# Autodesk Inventor assembly: Assembly2
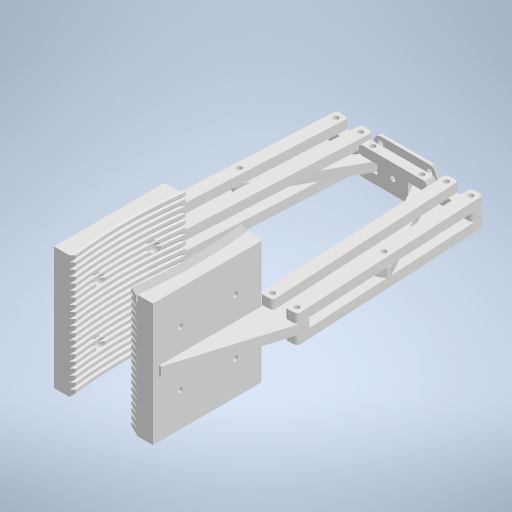
[picture p0: Inventor's stored thumbnail of the model, 512x512]
Saved by Autodesk Inventor 2023 (Build 270158000, 158)
## iProperties
Created: 2023-02-27
Part Number: Assembly2
Document SubType Name: Assembly
Designer: Gabriel - T3 CAD
Author: Gabriel - T3 CAD
## Documents named in this file (14)
- C:\Users\Gabriel - T3 CAD\Downloads\New folder\Assembly2.iam
- C:\Users\Gabriel - T3 CAD\Downloads\New folder\Outer swing.ipt
- C:\Users\Gabriel - T3 CAD\Downloads\New folder\Inner swing.ipt
- C:\Users\Gabriel - T3 CAD\Downloads\New folder\Pusher.ipt
- C:\Users\Gabriel - T3 CAD\Downloads\New folder\Connector.ipt
- C:\Users\Gabriel - T3 CAD\Downloads\New folder\Gripper triangle.ipt
- C:\Users\Gabriel - T3 CAD\Downloads\New folder\Gripper plate.ipt
- C:\Users\Gabriel - T3 CAD\Downloads\New folder\Outer swing_MIR.ipt
- C:\Users\Gabriel - T3 CAD\Downloads\New folder\Inner swing_MIR.ipt
- C:\Users\Gabriel - T3 CAD\Downloads\New folder\Pusher_MIR.ipt
- C:\Users\Gabriel - T3 CAD\Downloads\New folder\Gripper triangle_MIR.ipt
- C:\Users\Gabriel - T3 CAD\Downloads\New folder\Gripper plate_MIR.ipt
- C:\Users\Gabriel - T3 CAD\Downloads\New folder\Face Plate.ipt
- C:\Users\Gabriel - T3 CAD\Documents\GitHub\T3-CAD\Current Season CAD\Swerve-DriveTrain-V2.1 (LongBot)\Potential new gripper\Gripper plate v2.ipt
## Components (18 placed, 13 different names)
1. Outer swing:1 — Insert:1, Insert:7
2. Inner swing:1 — Insert:9, Insert:19
3. Pusher:1 — Insert:1, Insert:2, Insert:3
4. Outer swing:2 — Insert:2, Insert:8, Insert:23
5. Connector:1 — Insert:3, Insert:18, Insert:29
6. Inner swing:2 — Insert:10, Insert:20
7. Gripper triangle:1 — Rigid:1, Insert:7, Insert:8, Insert:9, Insert:10
8. Gripper plate:1 — Rigid:1, Insert:26, Insert:28
9. Outer swing_MIR:1 — Insert:11, Insert:17
10. Inner swing_MIR:1 — Insert:15, Insert:21
11. Pusher_MIR:1 — Insert:11, Insert:12, Insert:18
12. Outer swing_MIR:2 — Insert:12, Insert:16, Insert:24
13. Inner swing_MIR:2 — Insert:14, Insert:22
14. Gripper triangle_MIR:1 — Insert:14, Insert:15, Insert:16, Insert:17, Rigid:2
15. Gripper plate_MIR:1 — Rigid:2, Insert:25, Insert:27
16. Face Plate:1 — Insert:19, Insert:20, Insert:21, Insert:22, Insert:23, Insert:24, Insert:29
17. Gripper plate v2:1 — Insert:26, Insert:28
18. Gripper plate v2:2 — Insert:25, Insert:27
## Relationships (27: Insert 25, WeldJoint 2)
- Insert:1: Outer swing:1 ↔ Pusher:1
- Insert:2: Pusher:1 ↔ Outer swing:2
- Insert:3: Pusher:1 ↔ Connector:1
- Rigid:1 [WeldJoint]: Gripper triangle:1 ↔ Gripper plate:1
- Insert:7: Outer swing:1 ↔ Gripper triangle:1
- Insert:8: Outer swing:2 ↔ Gripper triangle:1
- Insert:9: Inner swing:1 ↔ Gripper triangle:1
- Insert:10: Inner swing:2 ↔ Gripper triangle:1
- Insert:11: Outer swing_MIR:1 ↔ Pusher_MIR:1
- Insert:12: Pusher_MIR:1 ↔ Outer swing_MIR:2
- Insert:14: Inner swing_MIR:2 ↔ Gripper triangle_MIR:1
- Insert:15: Inner swing_MIR:1 ↔ Gripper triangle_MIR:1
- Insert:16: Outer swing_MIR:2 ↔ Gripper triangle_MIR:1
- Insert:17: Outer swing_MIR:1 ↔ Gripper triangle_MIR:1
- Rigid:2 [WeldJoint]: Gripper triangle_MIR:1 ↔ Gripper plate_MIR:1
- Insert:18: Connector:1 ↔ Pusher_MIR:1
- Insert:19: Inner swing:1 ↔ Face Plate:1
- Insert:20: Inner swing:2 ↔ Face Plate:1
- Insert:21: Inner swing_MIR:1 ↔ Face Plate:1
- Insert:22: Inner swing_MIR:2 ↔ Face Plate:1
- Insert:23: Outer swing:2 ↔ Face Plate:1
- Insert:24: Outer swing_MIR:2 ↔ Face Plate:1
- Insert:25: Gripper plate_MIR:1 ↔ Gripper plate v2:2
- Insert:26: Gripper plate:1 ↔ Gripper plate v2:1
- Insert:27: Gripper plate_MIR:1 ↔ Gripper plate v2:2
- Insert:28: Gripper plate:1 ↔ Gripper plate v2:1
- Insert:29 (3.175 mm): Connector:1 ↔ Face Plate:1
